# Autodesk Inventor assembly: Hand Kwik-Mount
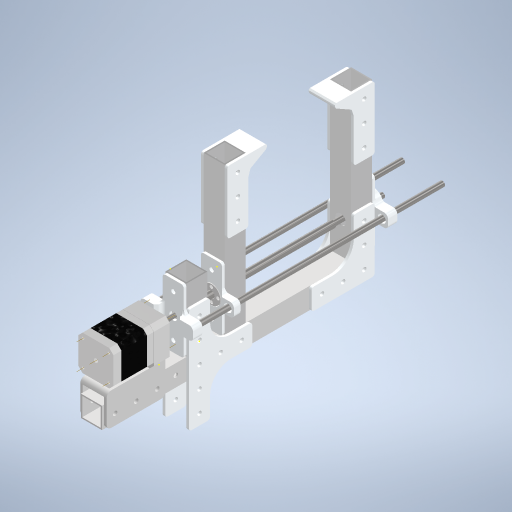
[picture p0: Inventor's stored thumbnail of the model, 512x512]
Saved by Autodesk Inventor 2024 (Build 280153000, 153)
## iProperties
Created: 2024-01-20
Part Number: Hand Kwik-Mount
Document SubType Name: Assembly
Designer: aidan
Author: aidan
## Documents named in this file (15)
- C:\Users\aidan\OneDrive\Documents\Inventor\Content Center Files\CH - Hand W Standard Gussets.iam
- C:\Users\aidan\OneDrive\Documents\Inventor\Content Center Files\am-4158 1IN Tee Gusset.ipt
- C:\Users\aidan\OneDrive\Documents\Inventor\Content Center Files\am-3860 90 Gusset REV2.ipt
- C:\Users\aidan\OneDrive\Documents\Inventor\Content Center Files\Tube Finger.ipt
- C:\Users\aidan\OneDrive\Documents\Inventor\Content Center Files\Lead Nut Holder Mk2.ipt
- C:\Users\aidan\OneDrive\Documents\Inventor\Content Center Files\Guide Rod Holder.ipt
- C:\Users\aidan\OneDrive\Documents\Inventor\Content Center Files\Finger Base.ipt
- C:\Users\aidan\OneDrive\Documents\Inventor\Content Center Files\Lead_Shaft.ipt
- C:\Users\aidan\OneDrive\Documents\Inventor\Content Center Files\Bearing Holder.ipt
- C:\Users\aidan\OneDrive\Documents\Inventor\Content Center Files\Guide Shaft.ipt
- C:\Users\aidan\OneDrive\Documents\Inventor\Content Center Files\Tube End.ipt
- C:\Users\aidan\OneDrive\Documents\Inventor\Content Center Files\Nema 17 stepper motor.ipt
- C:\Users\aidan\OneDrive\Documents\Inventor\Content Center Files\Arm Wedge Thingy.ipt
- C:\Users\aidan\OneDrive\Documents\Inventor\Content Center Files\Lead Nut.ipt
- C:\Users\aidan\OneDrive\Documents\Inventor\Content Center Files\Nema Mount.ipt
## Components (19 placed, 14 different names)
1. am-3860 90 Gusset REV2:1
2. am-3860 90 Gusset REV2:2 — Rotational:4
3. Tube Finger:2 — Rotational:20, Rotational:21
4. Lead Nut Holder Mk2:1
5. Finger Base:1 — Rotational:4, Rotational:5, Rotational:6, Rigid:1, Rotational:22
6. am-4158 1IN Tee Gusset:1 — Rotational:6
7. am-4158 1IN Tee Gusset:2 — Rotational:5
8. Guide Rod Holder:2 — Rotational:9, Rotational:17, Mate:2
9. Lead_Shaft:2 — Rotational:9
10. Bearing Holder:1
11. Guide Shaft:1 — Rotational:17
12. Guide Shaft:2 — Mate:2
13. Tube Finger:4 — Rigid:1, Rotational:19
14. Tube End:1
15. Nema 17 stepper motor:1
16. Arm Wedge Thingy:1 — Rotational:20
17. Arm Wedge Thingy:2 — Rotational:19
18. Lead Nut:1 — Rotational:21
19. Nema Mount:1 — Rotational:22
## Relationships (11: RevoluteJoint 9, Mate 1, WeldJoint 1)
- Rotational:4 [RevoluteJoint]: am-3860 90 Gusset REV2:2 ↔ Finger Base:1
- Rotational:5 [RevoluteJoint]: Finger Base:1 ↔ am-4158 1IN Tee Gusset:2
- Rotational:6 [RevoluteJoint]: Finger Base:1 ↔ am-4158 1IN Tee Gusset:1
- Rotational:9 [RevoluteJoint] (-12.7 mm): Guide Rod Holder:2 ↔ Lead_Shaft:2
- Rotational:17 [RevoluteJoint]: Guide Rod Holder:2 ↔ Guide Shaft:1
- Mate:2: Guide Rod Holder:2 ↔ Guide Shaft:2
- Rigid:1 [WeldJoint]: Finger Base:1 ↔ Tube Finger:4
- Rotational:19 [RevoluteJoint]: Tube Finger:4 ↔ Arm Wedge Thingy:2
- Rotational:20 [RevoluteJoint]: Tube Finger:2 ↔ Arm Wedge Thingy:1
- Rotational:21 [RevoluteJoint]: Tube Finger:2 ↔ Lead Nut:1
- Rotational:22 [RevoluteJoint]: Finger Base:1 ↔ Nema Mount:1
